# Autodesk Inventor assembly: !drive-pod
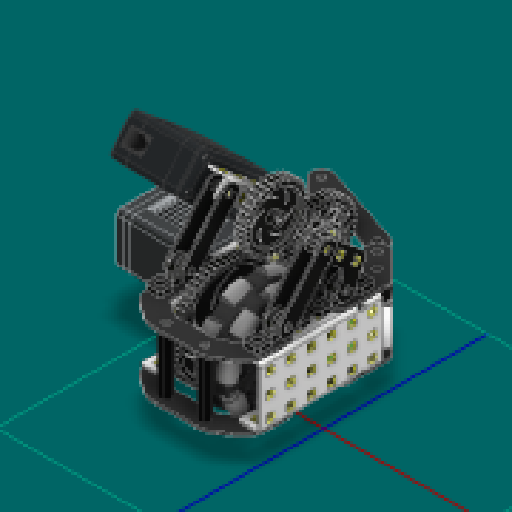
[picture p0: Inventor's stored thumbnail of the model, 512x512]
Saved by Autodesk Inventor 2025 (Build 290162000, 162)
## iProperties
Created: 2024-08-10
Part Number: !drive-pod
Document SubType Name: Assembly
Designer: averey
Author: averey
## Documents named in this file (26)
- C:\Users\avere\rbp_cad\atlas\chassis\drive-pod\!drive-pod.iam
- C:\Users\avere\rbp_cad\VEX-CAD-Inventor-1.41\Structure\C Channel\Aluminum 1x3x1\Alu C 1x3x1x6.ipt
- C:\Users\avere\rbp_cad\VEX-CAD-Inventor-1.41\Structure\Standoff\Standoff 1.50.ipt
- C:\Users\avere\rbp_cad\VEX-CAD-Inventor-1.41\Structure\Standoff.ipt
- C:\Users\avere\rbp_cad\VEX-CAD-Inventor-1.41\Motion\Shaft LS\LS Pillow Bearing Block.ipt
- C:\Users\avere\rbp_cad\VEX-CAD-Inventor-1.41\Structure\C Channel\Aluminum 1x3x1\Alu C 1x3x1x8.ipt
- C:\Users\avere\rbp_cad\atlas\chassis\drive-pod\custom-parts\gearbox-support-gusset.ipt
- C:\Users\avere\rbp_cad\atlas\chassis\drive-pod\custom-parts\gearbox-gusset.ipt
- C:\Users\avere\rbp_cad\VEX-CAD-Inventor-1.41\Motion\Shaft LS\Bearing Flat Low Profile.ipt
- C:\Users\avere\rbp_cad\VEX-CAD-Inventor-1.41\Structure\Angle\Aluminum 1x1\Alu Angle 1x1x5.ipt
- C:\Users\avere\rbp_cad\VEX-CAD-Inventor-1.41\Electronics\Motors with Screws\SteelM-StarS.iam
- C:\Users\avere\rbp_cad\VEX-CAD-Inventor-1.41\Electronics\Motors with Screws.iam
- C:\Users\avere\rbp_cad\VEX-CAD-Inventor-1.41\Electronics\V5 Motor (5.5W).ipt
- C:\Users\avere\rbp_cad\atlas\chassis\drive-pod\custom-parts\elbow-gusset.ipt
- C:\Users\avere\rbp_cad\VEX-CAD-Inventor-1.41\Motion\Gears\LS 36T Gear.ipt
- C:\Users\avere\rbp_cad\VEX-CAD-Inventor-1.41\Motion\Gears\LS 60T Gear.ipt
- C:\Users\avere\rbp_cad\VEX-CAD-Inventor-1.41\Motion\Wheels\Omni Wheel\2.75 Omni AS, No Insert.iam
- C:\Users\avere\rbp_cad\VEX-CAD-Inventor-1.41\Motion\Wheels\Omni Wheel.iam
- C:\Users\avere\rbp_cad\VEX-CAD-Inventor-1.41\Motion\Gears\LS 12T Gear.ipt
- C:\Users\avere\rbp_cad\atlas\chassis\drive-pod\custom-parts\half_cut_36t.ipt
- C:\Users\avere\rbp_cad\VEX-CAD-Inventor-1.41\Structure\C Channel\Aluminum 1x2x1\Alu C 1x2x1x3.ipt
- C:\Users\avere\rbp_cad\atlas\chassis\drive-pod\custom-parts\join-gusset_offset.ipt
- C:\Users\avere\rbp_cad\VEX-CAD-Inventor-1.41\Motion\Spacers\Spacer Nylon .500 OD\NSpacer Black .500 OD x .500.ipt
- C:\Users\avere\rbp_cad\VEX-CAD-Inventor-1.41\Motion\Spacers\Spacer Nylon .500 OD.ipt
- C:\Users\avere\rbp_cad\VEX-CAD-Inventor-1.41\Motion\Spacers\Spacer Nylon .500 OD\NSpacer Black .500 OD x .375.ipt
- C:\Users\avere\rbp_cad\atlas\chassis\drive-pod\custom-parts\funnel_gusset_full.ipt
## Components (36 placed, 21 different names)
1. Alu C 1x3x1x6:1 — Mate:4, Insert:7, Mate:5, Insert:34, Mate:24, Insert:36, Mate:26, Insert:50, Mate:31
2. Standoff 1.50:1 — Insert:47
3. Standoff 1.50:2 — Insert:46
4. LS Pillow Bearing Block:1 — Mate:4, Mate:7, Insert:11
5. LS Pillow Bearing Block:2 — Insert:7, Mate:5, Insert:9, Mate:8
6. Alu C 1x3x1x8:1 — Mate:10, Insert:15, Mate:11, Insert:20, Mate:15, Insert:26, Insert:27, Insert:37, Mate:27, Mate:28, Mate:29, Mate:30, Insert:48, Insert:49
7. gearbox-support-gusset:1 — Insert:9, Insert:10, Insert:13
8. gearbox-gusset:1 — Mate:7, Insert:10, Mate:9
9. gearbox-support-gusset:2 — Insert:12, Mate:8
10. gearbox-gusset:2 — Insert:11, Insert:12
11. Bearing Flat Low Profile:1 — Insert:13, Mate:9
12. LS Pillow Bearing Block:3 — Mate:10, Insert:17, Insert:18
13. LS Pillow Bearing Block:4 — Insert:15, Mate:11, Insert:16
14. Alu Angle 1x1x5:1 — Insert:16, Mate:12, Mate:13, Insert:30, Insert:31, Mate:22, Insert:32
15. gearbox-gusset:3 — Insert:17, Mate:12
16. gearbox-gusset:4 — Insert:18, Mate:13
17. SteelM-StarS:1 [sub-assembly] — Insert:20, Mate:15
18. V5 Motor (5.5W):1 — Insert:31, Mate:22
19. LS 36T Gear:1 — Insert:26, Insert:29
20. LS 60T Gear:1 — Insert:27, Insert:28, Mate:21
21. 2.75 Omni AS, No Insert:1 [sub-assembly] — Insert:28, Mate:21
22. LS 12T Gear:1 — Insert:29
23. half_cut_36t:1 — Insert:30
24. LS 36T Gear:3 — Insert:32
25. elbow-gusset:2 — Insert:34, Mate:24, Insert:35, Mate:25
26. Alu C 1x2x1x3:1 — Insert:35, Mate:25, Insert:38, Insert:41
27. elbow-gusset:3 — Insert:36, Mate:26, Insert:39, Insert:40
28. join-gusset_offset:1 — Insert:37, Mate:27, Insert:43, Insert:44
29. join-gusset_offset:2 — Insert:38, Mate:28
30. NSpacer Black .500 OD x .500:1 — Insert:39
31. NSpacer Black .500 OD x .500:2 — Insert:40
32. NSpacer Black .500 OD x .375:3 — Insert:41
33. NSpacer Black .500 OD x .375:4 — Insert:43
34. NSpacer Black .500 OD x .375:5 — Insert:44
35. funnel_gusset_full:1 — Mate:29, Insert:46, Insert:47, Insert:49, Insert:50, Mate:31
36. funnel_gusset_full:2 — Mate:30, Insert:48
## Relationships (53: Insert 33, Mate 20)
- Mate:4: Alu C 1x3x1x6:1 ↔ LS Pillow Bearing Block:1
- Insert:7 (3.175 mm): Alu C 1x3x1x6:1 ↔ LS Pillow Bearing Block:2
- Mate:5: Alu C 1x3x1x6:1 ↔ LS Pillow Bearing Block:2
- Insert:9: LS Pillow Bearing Block:2 ↔ gearbox-support-gusset:1
- Mate:7: LS Pillow Bearing Block:1 ↔ gearbox-gusset:1
- Insert:10: gearbox-support-gusset:1 ↔ gearbox-gusset:1
- Insert:11: LS Pillow Bearing Block:1 ↔ gearbox-gusset:2
- Insert:12: gearbox-support-gusset:2 ↔ gearbox-gusset:2
- Mate:8: LS Pillow Bearing Block:2 ↔ gearbox-support-gusset:2
- Insert:13: gearbox-support-gusset:1 ↔ Bearing Flat Low Profile:1
- Mate:9: gearbox-gusset:1 ↔ Bearing Flat Low Profile:1
- Mate:10: Alu C 1x3x1x8:1 ↔ LS Pillow Bearing Block:3
- Insert:15: Alu C 1x3x1x8:1 ↔ LS Pillow Bearing Block:4
- Mate:11: Alu C 1x3x1x8:1 ↔ LS Pillow Bearing Block:4
- Insert:16: LS Pillow Bearing Block:4 ↔ Alu Angle 1x1x5:1
- Insert:17 (1.5875 mm): LS Pillow Bearing Block:3 ↔ gearbox-gusset:3
- Mate:12: Alu Angle 1x1x5:1 ↔ gearbox-gusset:3
- Insert:18: LS Pillow Bearing Block:3 ↔ gearbox-gusset:4
- Mate:13: Alu Angle 1x1x5:1 ↔ gearbox-gusset:4
- Insert:20: Alu C 1x3x1x8:1 ↔ SteelM-StarS:1
- Mate:15: Alu C 1x3x1x8:1 ↔ SteelM-StarS:1
- Insert:26 (0.3969 mm): Alu C 1x3x1x8:1 ↔ LS 36T Gear:1
- Insert:27 (0.3969 mm): Alu C 1x3x1x8:1 ↔ LS 60T Gear:1
- Insert:28 (19.05 mm): LS 60T Gear:1 ↔ 2.75 Omni AS, No Insert:1
- Mate:21: LS 60T Gear:1 ↔ 2.75 Omni AS, No Insert:1
- Insert:29: LS 36T Gear:1 ↔ LS 12T Gear:1
- Insert:30 (11.5094 mm): Alu Angle 1x1x5:1 ↔ half_cut_36t:1
- Insert:31: Alu Angle 1x1x5:1 ↔ V5 Motor (5.5W):1
- Mate:22: Alu Angle 1x1x5:1 ↔ V5 Motor (5.5W):1
- Insert:32 (12.7 mm): Alu Angle 1x1x5:1 ↔ LS 36T Gear:3
- Insert:34: Alu C 1x3x1x6:1 ↔ elbow-gusset:2
- Mate:24: Alu C 1x3x1x6:1 ↔ elbow-gusset:2
- Insert:35: elbow-gusset:2 ↔ Alu C 1x2x1x3:1
- Mate:25: elbow-gusset:2 ↔ Alu C 1x2x1x3:1
- Insert:36: Alu C 1x3x1x6:1 ↔ elbow-gusset:3
- Mate:26: Alu C 1x3x1x6:1 ↔ elbow-gusset:3
- Insert:37: Alu C 1x3x1x8:1 ↔ join-gusset_offset:1
- Mate:27: Alu C 1x3x1x8:1 ↔ join-gusset_offset:1
- Insert:38: Alu C 1x2x1x3:1 ↔ join-gusset_offset:2
- Mate:28: Alu C 1x3x1x8:1 ↔ join-gusset_offset:2
- Insert:39: elbow-gusset:3 ↔ NSpacer Black .500 OD x .500:1
- Insert:40: elbow-gusset:3 ↔ NSpacer Black .500 OD x .500:2
- Insert:41: Alu C 1x2x1x3:1 ↔ NSpacer Black .500 OD x .375:3
- Insert:43: join-gusset_offset:1 ↔ NSpacer Black .500 OD x .375:4
- Insert:44: join-gusset_offset:1 ↔ NSpacer Black .500 OD x .375:5
- Mate:29: Alu C 1x3x1x8:1 ↔ funnel_gusset_full:1
- Insert:46: Standoff 1.50:2 ↔ funnel_gusset_full:1
- Insert:47: Standoff 1.50:1 ↔ funnel_gusset_full:1
- Mate:30: Alu C 1x3x1x8:1 ↔ funnel_gusset_full:2
- Insert:48: Alu C 1x3x1x8:1 ↔ funnel_gusset_full:2
- Insert:49: Alu C 1x3x1x8:1 ↔ funnel_gusset_full:1
- Insert:50: Alu C 1x3x1x6:1 ↔ funnel_gusset_full:1
- Mate:31: Alu C 1x3x1x6:1 ↔ funnel_gusset_full:1
